# Autodesk Inventor assembly: Assembly_HoLiSheet_v1
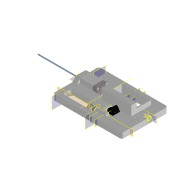
[picture p0: Inventor's stored thumbnail of the model, 180x180]
Saved by Autodesk Inventor 2022 (Build 260153000, 153)
## iProperties
Created: 2022-09-27
Part Number: Assembly_HoLiSheet_v1
Document SubType Name: Assembly
Designer: UC2
Author: UC2
## Documents named in this file (8)
- C:\Users\diederichbenedict\Dropbox\Dokumente\Promotion\PROJECTS\HoLiSheet\INVENTOR\Assembly_HoLiSheet_v1.iam
- C:\Users\diederichbenedict\Dropbox\Dokumente\Promotion\PROJECTS\HoLiSheet\INVENTOR\Assembly_HoLiSheet_TwoHalf_v1.iam
- C:\Users\diederichbenedict\Dropbox\Dokumente\Promotion\PROJECTS\HoLiSheet\INVENTOR\00_CCTV_lens_M12_25mm_5mp.ipt
- C:\Users\diederichbenedict\Dropbox\Dokumente\Promotion\PROJECTS\HoLiSheet\INVENTOR\00_PipetteTip200ul-1.ipt
- C:\Users\diederichbenedict\Dropbox\Dokumente\Promotion\PROJECTS\HoLiSheet\INVENTOR\00_FEP_tube_2.2x0.5mm.ipt
- C:\Users\diederichbenedict\Dropbox\Dokumente\Promotion\PROJECTS\HoLiSheet\INVENTOR\00_NEMA8.ipt
- C:\Users\diederichbenedict\Dropbox\Dokumente\Promotion\PROJECTS\HoLiSheet\INVENTOR\00_huawei_p30_Objectivelensassembly.ipt
- C:\Users\diederichbenedict\Dropbox\Dokumente\Promotion\PROJECTS\HoLiSheet\INVENTOR\20_SMAConnector_fiber.ipt
## Components (8 placed, 7 different names)
1. Assembly_HoLiSheet_TwoHalf_v1:1 [sub-assembly] — Einfügen:1, Einfügen:2, Tangential:1, Passend:4, Winkel:1, Passend:5, Einfügen:3, Fluchtend:2
2. 00_CCTV_lens_M12_25mm_5mp:1 — Tangential:1, Einfügen:3, Passend:6
3. 00_PipetteTip200ul-1:1
4. 00_FEP_tube_2.2x0.5mm:1
5. 00_PipetteTip200ul-1:2 — Einfügen:2
6. 00_NEMA8:1 — Einfügen:1
7. 00_huawei_p30_Objectivelensassembly:1 — Passend:6, Fluchtend:2, Einfügen:4
8. 20_SMAConnector_fiber:1 — Einfügen:4
## Relationships (13: Mate 6, Insert 4, Tangent 1, Angle 1, Flush 1)
- [Mate]: 00_FEP_tube_2.2x0.5mm:1 ↔ 00_PipetteTip200ul-1:2
- [Mate]: 00_PipetteTip200ul-1:1 ↔ 00_FEP_tube_2.2x0.5mm:1
- [Mate]: 00_CCTV_lens_M12_25mm_5mp:1 ↔ 00_PipetteTip200ul-1:2
- Einfügen:1 [Insert]: Assembly_HoLiSheet_TwoHalf_v1:1 ↔ 00_NEMA8:1
- Einfügen:2 [Insert]: Assembly_HoLiSheet_TwoHalf_v1:1 ↔ 00_PipetteTip200ul-1:2
- Tangential:1: Assembly_HoLiSheet_TwoHalf_v1:1 ↔ 00_CCTV_lens_M12_25mm_5mp:1
- Passend:4 [Mate]: Assembly_HoLiSheet_TwoHalf_v1:1
- Winkel:1 [Angle] (0 deg): Assembly_HoLiSheet_TwoHalf_v1:1
- Passend:5 [Mate]: Assembly_HoLiSheet_TwoHalf_v1:1
- Einfügen:3 [Insert]: Assembly_HoLiSheet_TwoHalf_v1:1 ↔ 00_CCTV_lens_M12_25mm_5mp:1
- Passend:6 [Mate]: 00_CCTV_lens_M12_25mm_5mp:1 ↔ 00_huawei_p30_Objectivelensassembly:1
- Fluchtend:2 [Flush]: Assembly_HoLiSheet_TwoHalf_v1:1 ↔ 00_huawei_p30_Objectivelensassembly:1
- Einfügen:4 [Insert] (2 mm): 00_huawei_p30_Objectivelensassembly:1 ↔ 20_SMAConnector_fiber:1
